# Autodesk Inventor assembly: stepper_motor
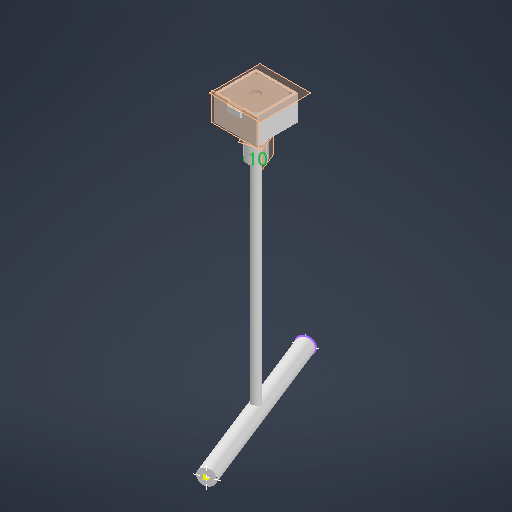
[picture p0: Inventor's stored thumbnail of the model, 512x512]
Saved by Autodesk Inventor 2025.2 (Build 292293000, 293)
## iProperties
Created: 2024-11-23
Part Number: stepper_motor
Document SubType Name: Assembly
Designer: dell
Author: dell
## Documents named in this file (5)
- C:\Users\ktamu\LocalLenovoKei\CrepeLocal\CAD2\CAD\Tonbo.iam
- C:\Users\ktamu\LocalLenovoKei\CrepeLocal\CAD2\CAD\joint.ipt
- C:\Users\ktamu\LocalLenovoKei\CrepeLocal\CAD2\CAD\Tonbo.ipt
- C:\Users\ktamu\LocalLenovoKei\CrepeLocal\CAD2\CAD\stepper_motor.ipt
- C:\Users\ktamu\LocalLenovoKei\CrepeLocal\CAD2\CAD\motor_case.ipt
## Components (4 placed, 4 different names)
1. joint:1 — 回転:1, 挿入:2, 回転:1
2. Tonbo:1 — 挿入:2, 回転:1
3. stepper_motor:1 — 回転:1, 挿入:1
4. motor_case:1 — 挿入:1
## Relationships (4: Insert 2, RevoluteJoint 1, RelateRotation 1)
- 回転:1 [RevoluteJoint]: joint:1 ↔ stepper_motor:1
- 挿入:1 [Insert]: stepper_motor:1 ↔ motor_case:1
- 挿入:2 [Insert]: joint:1 ↔ Tonbo:1
- 回転:1 [RelateRotation] (1 ul): joint:1 ↔ Tonbo:1
